# Autodesk Inventor assembly: intake
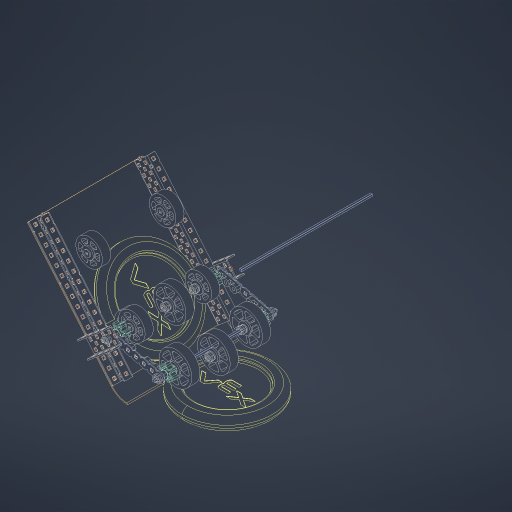
[picture p0: Inventor's stored thumbnail of the model, 512x512]
Saved by Autodesk Inventor 2023 (Build 270158000, 158)
## iProperties
Created: 2023-02-25
Part Number: intake
Document SubType Name: Assembly
Designer: Windows Macbook
Author: Windows Macbook
## Documents named in this file (19)
- C:\Users\Windows Macbook\Desktop\VRC-SPIN-UP\Inventor\Assembly\Pre Worlds\intake.iam
- C:\Users\Windows Macbook\Desktop\VRC-SPIN-UP\Inventor\Custom\intakeabs.ipt
- C:\Users\Windows Macbook\Desktop\VRC-SPIN-UP\Inventor\Disk.ipt
- C:\Users\Windows Macbook\Desktop\VRC-SPIN-UP\Inventor\Structure\Standoff.ipt
- C:\Users\Windows Macbook\Desktop\VRC-SPIN-UP\Inventor\Motion\Wheels\Flex Wheels\2 Flex, LS.iam
- C:\Users\Windows Macbook\Desktop\VRC-SPIN-UP\Inventor\Motion\Wheels\Flex Wheels\1.625 Flex, LS.iam
- C:\Users\Windows Macbook\Desktop\VRC-SPIN-UP\Inventor\Structure\C Channel\Aluminum 1x2x1\Alu C 1x2x1x16.ipt
- C:\Users\Windows Macbook\Desktop\VRC-SPIN-UP\Inventor\Structure\Standoff\Standoff .50.ipt
- C:\Users\Windows Macbook\Desktop\VRC-SPIN-UP\Inventor\Motion\Spacers\Spacer Nylon .313 OD\NSpacer .313 OD x .125.ipt
- C:\Users\Windows Macbook\Desktop\VRC-SPIN-UP\Inventor\Motion\Spacers\Spacer Nylon .313 OD.ipt
- C:\Users\Windows Macbook\Desktop\VRC-SPIN-UP\Inventor\Motion\Shaft LS\Bearing Flat.ipt
- C:\Users\Windows Macbook\Desktop\VRC-SPIN-UP\Inventor\Motion\Shaft LS\Shaft LS.ipt
- C:\Users\Windows Macbook\Desktop\VRC-SPIN-UP\Inventor\Motion\Shaft LS\Shaft Collar Rubber.ipt
- C:\Users\Windows Macbook\Desktop\VRC-SPIN-UP\Inventor\Motion\Shaft LS\Shaft LS\Shaft LS 7.5.ipt
- C:\Users\Windows Macbook\Desktop\VRC-SPIN-UP\Inventor\Motion\Sprockets\9P Sprocket\9P 6T Sprocket, Square.iam
- C:\Users\Windows Macbook\Desktop\VRC-SPIN-UP\Inventor\Motion\Sprockets\9P Sprocket.iam
- C:\Users\Windows Macbook\Desktop\VRC-SPIN-UP\Inventor\Motion\Shaft LS\Shaft LS\Shaft LS 8.0.ipt
- C:\Users\Windows Macbook\Desktop\VRC-SPIN-UP\Inventor\Structure\C Channel\Aluminum 1x2x1\Alu C 1x2x1x4.ipt
- C:\Users\Windows Macbook\Desktop\VRC-SPIN-UP\Inventor\Structure\Plate\Steel\Steel Plate 1x7.ipt
## Components (47 placed, 14 different names)
1. intakeabs:1 — Insert:5, Insert:6, Insert:7, Insert:8
2. Disk:1
3. Disk:2
4. 1.625 Flex, LS:1 [sub-assembly] — Insert:56
5. 1.625 Flex, LS:2 [sub-assembly] — Insert:57, Insert:73
6. 1.625 Flex, LS:3 [sub-assembly]
7. 1.625 Flex, LS:4 [sub-assembly]
8. 2 Flex, LS:5 [sub-assembly] — Insert:47, Insert:48
9. 2 Flex, LS:6 [sub-assembly] — Insert:45, Insert:77
10. Alu C 1x2x1x16:1 — Insert:5, Insert:6, Insert:13, Insert:15
11. Alu C 1x2x1x16:2 — Insert:7, Insert:8, Insert:25, Insert:26
12. Alu C 1x2x1x4:1 — Insert:86, Insert:92
13. Standoff .50:2 — Insert:15
14. Standoff .50:3 — Insert:13
15. Standoff .50:4 — Insert:25, Insert:69
16. Standoff .50:5 — Insert:26
17. Alu C 1x2x1x4:2 — Insert:66, Insert:69, Insert:90
18. Shaft Collar Rubber:5 — Insert:45
19. Shaft Collar Rubber:8 — Insert:48
20. Shaft Collar Rubber:9 — Insert:47
21. 2 Flex, LS:7 [sub-assembly]
22. Shaft Collar Rubber:10 — Insert:58
23. Shaft Collar Rubber:11
24. Shaft Collar Rubber:12 — Insert:56, Insert:58
25. Shaft Collar Rubber:13 — Insert:57
26. Steel Plate 1x7:1 — Insert:70, Insert:71, Insert:75, Insert:76, Insert:91
27. NSpacer .313 OD x .125:8 — Insert:66
28. Bearing Flat:5 — Insert:70, Insert:71, Insert:72
29. 9P 6T Sprocket, Square:3 [sub-assembly] — Insert:72, Insert:73
30. Bearing Flat:6 — Insert:75, Insert:76
31. 9P 6T Sprocket, Square:4 [sub-assembly] — Insert:77
32. 1.625 Flex, LS:5 [sub-assembly]
33. 2 Flex, LS:8 [sub-assembly]
34. Shaft Collar Rubber:14
35. Shaft Collar Rubber:15
36. NSpacer .313 OD x .125:9 — Insert:86
37. Steel Plate 1x7:2 — Insert:87, Insert:88, Insert:93
38. Bearing Flat:7
39. 9P 6T Sprocket, Square:5 [sub-assembly]
40. 9P 6T Sprocket, Square:6 [sub-assembly] — Insert:89
41. Bearing Flat:8 — Insert:87, Insert:88, Insert:89
42. Shaft LS 7.5:3 — Flush:1, Cylindrical:1
43. Shaft LS 8.0:4
44. Shaft Collar Rubber:16 — Insert:91, Flush:1, Cylindrical:1
45. Shaft Collar Rubber:17 — Insert:90
46. Shaft Collar Rubber:18 — Insert:93
47. Shaft Collar Rubber:19 — Insert:92
## Relationships (48: Insert 44, Angle 2, Flush 1, CylindricalJoint 1)
- Insert:5: intakeabs:1 ↔ Alu C 1x2x1x16:1
- Insert:6: intakeabs:1 ↔ Alu C 1x2x1x16:1
- Insert:7: intakeabs:1 ↔ Alu C 1x2x1x16:2
- Insert:8: intakeabs:1 ↔ Alu C 1x2x1x16:2
- Insert:13: Alu C 1x2x1x16:1 ↔ Standoff .50:3
- [Insert]: Alu C 1x2x1x4:1 ↔ Standoff .50:3
- [Angle] (0 deg): intakeabs:1 ↔ Alu C 1x2x1x4:1
- Insert:15: Alu C 1x2x1x16:1 ↔ Standoff .50:2
- Insert:25: Alu C 1x2x1x16:2 ↔ Standoff .50:4
- Insert:26: Alu C 1x2x1x16:2 ↔ Standoff .50:5
- [Angle] (0 deg): intakeabs:1 ↔ Alu C 1x2x1x4:2
- Insert:45 (0.889 mm): 2 Flex, LS:6 ↔ Shaft Collar Rubber:5
- Insert:47 (0.889 mm): 2 Flex, LS:5 ↔ Shaft Collar Rubber:9
- Insert:48 (0.889 mm): 2 Flex, LS:5 ↔ Shaft Collar Rubber:8
- [Insert] (0.889 mm): 2 Flex, LS:7 ↔ Shaft Collar Rubber:11
- [Insert] (0.889 mm): 2 Flex, LS:7 ↔ Shaft Collar Rubber:10
- Insert:56 (0.889 mm): 1.625 Flex, LS:1 ↔ Shaft Collar Rubber:12
- Insert:57 (0.889 mm): 1.625 Flex, LS:2 ↔ Shaft Collar Rubber:13
- Insert:58 (27.94 mm): Shaft Collar Rubber:10 ↔ Shaft Collar Rubber:12
- [Insert]: Steel Plate 1x7:1 ↔ NSpacer .313 OD x .125:8
- Insert:66: Alu C 1x2x1x4:2 ↔ NSpacer .313 OD x .125:8
- Insert:69: Standoff .50:4 ↔ Alu C 1x2x1x4:2
- Insert:70: Steel Plate 1x7:1 ↔ Bearing Flat:5
- Insert:71: Steel Plate 1x7:1 ↔ Bearing Flat:5
- Insert:72: Bearing Flat:5 ↔ 9P 6T Sprocket, Square:3
- Insert:73: 1.625 Flex, LS:2 ↔ 9P 6T Sprocket, Square:3
- [Insert]: Bearing Flat:6 ↔ 9P 6T Sprocket, Square:4
- Insert:75: Steel Plate 1x7:1 ↔ Bearing Flat:6
- Insert:76: Steel Plate 1x7:1 ↔ Bearing Flat:6
- Insert:77: 2 Flex, LS:6 ↔ 9P 6T Sprocket, Square:4
- [Insert] (0.889 mm): 2 Flex, LS:8 ↔ Shaft Collar Rubber:14
- [Insert] (0.889 mm): 1.625 Flex, LS:5 ↔ Shaft Collar Rubber:15
- [Insert]: NSpacer .313 OD x .125:9 ↔ Steel Plate 1x7:2
- [Insert]: Steel Plate 1x7:2 ↔ Bearing Flat:7
- [Insert]: Steel Plate 1x7:2 ↔ Bearing Flat:7
- [Insert]: Bearing Flat:7 ↔ 9P 6T Sprocket, Square:5
- [Insert]: 1.625 Flex, LS:5 ↔ 9P 6T Sprocket, Square:5
- [Insert]: 2 Flex, LS:8 ↔ 9P 6T Sprocket, Square:6
- Insert:86: Alu C 1x2x1x4:1 ↔ NSpacer .313 OD x .125:9
- Insert:87: Steel Plate 1x7:2 ↔ Bearing Flat:8
- Insert:88: Steel Plate 1x7:2 ↔ Bearing Flat:8
- Insert:89: 9P 6T Sprocket, Square:6 ↔ Bearing Flat:8
- Insert:90 (0.889 mm): Alu C 1x2x1x4:2 ↔ Shaft Collar Rubber:17
- Insert:91 (0.889 mm): Steel Plate 1x7:1 ↔ Shaft Collar Rubber:16
- Insert:92 (0.889 mm): Alu C 1x2x1x4:1 ↔ Shaft Collar Rubber:19
- Insert:93 (0.889 mm): Steel Plate 1x7:2 ↔ Shaft Collar Rubber:18
- Flush:1 (-3.175 mm): Shaft LS 7.5:3 ↔ Shaft Collar Rubber:16
- Cylindrical:1: Shaft LS 7.5:3 ↔ Shaft Collar Rubber:16
## Named parameters: d75_d68 = 0.889 mm, d76_d69 = 0.889 mm, d100_d98 = 0 mm, d104_d89 = 0 mm, d105_d78 = 0.889 mm, d106_d66 = 0.889 mm, d107_d95 = 0 mm, d108_d96 = 0 mm, d109_d98 = 0 mm, d110_d99 = 0 mm, d111_d103 = 0 mm
